# Autodesk Inventor assembly: Touch Segment
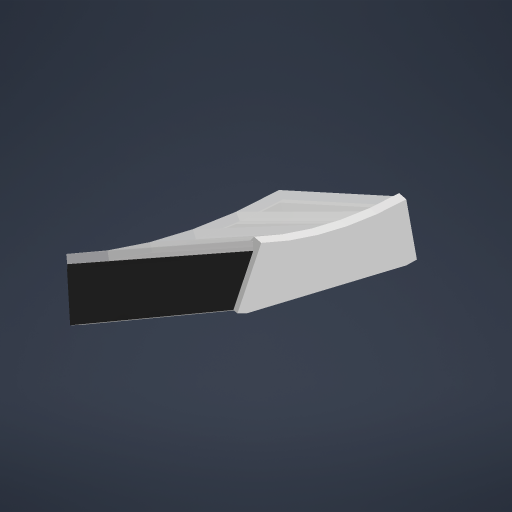
[picture p0: Inventor's stored thumbnail of the model, 512x512]
Saved by Autodesk Inventor 2023 (Build 270158000, 158)
## iProperties
Created: 2022-06-12
Part Number: Touch Segment
Document SubType Name: Assembly
Designer: FizzyApple12
Author: FizzyApple12
## Documents named in this file (4)
- C:\Users\FizzyApple12\Desktop\Wacca Controller\Touch Segment\Touch Segment.iam
- C:\Users\FizzyApple12\Desktop\Wacca Controller\Touch Segment\Touch Fifth.ipt
- C:\Users\FizzyApple12\Desktop\Wacca Controller\Touch Segment\Touch Casing.ipt
- C:\Users\FizzyApple12\Desktop\Wacca Controller\Touch Segment\Touch Segment Cover.ipt
## Components (7 placed, 3 different names)
1. Touch Fifth:1 — Mate:1, Mate:5, Flush:6, Mate:19, Mate:22, Mate:25, Mate:26, Flush:7, Flush:14
2. Touch Fifth:2 — Mate:1, Mate:2, Mate:5, Mate:6, Flush:5, Mate:16, Mate:18, Mate:20, Mate:21, Flush:13
3. Touch Fifth:3 — Mate:2, Mate:3, Mate:6, Mate:7, Mate:8, Flush:1, Flush:2, Mate:13, Mate:15, Mate:17, Flush:12
4. Touch Fifth:4 — Mate:3, Mate:4, Mate:7, Flush:3, Mate:9, Mate:11, Mate:12, Mate:14, Flush:11
5. Touch Fifth:5 — Mate:4, Mate:8, Flush:4, Mate:10, Mate:23, Mate:24, Flush:10
6. Touch Casing:1 — Flush:1, Flush:2, Flush:3, Flush:4, Flush:5, Flush:6, Mate:9, Mate:10, Mate:11, Mate:12, Mate:13, Mate:14, Mate:15, Mate:16, Mate:17, Mate:18, Mate:19, Mate:20, Mate:21, Mate:22, Mate:23, Mate:24, Mate:25, Mate:26, Flush:7, Flush:8, Flush:9
7. Touch Segment Cover:1 — Flush:8, Flush:9, Flush:10, Flush:11, Flush:12, Flush:13, Flush:14
## Relationships (40: Mate 26, Flush 14)
- Mate:1: Touch Fifth:1 ↔ Touch Fifth:2
- Mate:2: Touch Fifth:2 ↔ Touch Fifth:3
- Mate:3: Touch Fifth:3 ↔ Touch Fifth:4
- Mate:4: Touch Fifth:4 ↔ Touch Fifth:5
- Mate:5: Touch Fifth:1 ↔ Touch Fifth:2
- Mate:6: Touch Fifth:2 ↔ Touch Fifth:3
- Mate:7: Touch Fifth:3 ↔ Touch Fifth:4
- Mate:8: Touch Fifth:3 ↔ Touch Fifth:5
- Flush:1: Touch Fifth:3 ↔ Touch Casing:1
- Flush:2: Touch Fifth:3 ↔ Touch Casing:1
- Flush:3: Touch Fifth:4 ↔ Touch Casing:1
- Flush:4: Touch Fifth:5 ↔ Touch Casing:1
- Flush:5: Touch Fifth:2 ↔ Touch Casing:1
- Flush:6: Touch Fifth:1 ↔ Touch Casing:1
- Mate:9: Touch Fifth:4 ↔ Touch Casing:1
- Mate:10: Touch Fifth:5 ↔ Touch Casing:1
- Mate:11: Touch Fifth:4 ↔ Touch Casing:1
- Mate:12: Touch Fifth:4 ↔ Touch Casing:1
- Mate:13: Touch Fifth:3 ↔ Touch Casing:1
- Mate:14: Touch Fifth:4 ↔ Touch Casing:1
- Mate:15: Touch Fifth:3 ↔ Touch Casing:1
- Mate:16: Touch Fifth:2 ↔ Touch Casing:1
- Mate:17: Touch Fifth:3 ↔ Touch Casing:1
- Mate:18: Touch Fifth:2 ↔ Touch Casing:1
- Mate:19: Touch Fifth:1 ↔ Touch Casing:1
- Mate:20: Touch Fifth:2 ↔ Touch Casing:1
- Mate:21: Touch Fifth:2 ↔ Touch Casing:1
- Mate:22: Touch Fifth:1 ↔ Touch Casing:1
- Mate:23: Touch Fifth:5 ↔ Touch Casing:1
- Mate:24: Touch Fifth:5 ↔ Touch Casing:1
- Mate:25: Touch Fifth:1 ↔ Touch Casing:1
- Mate:26: Touch Fifth:1 ↔ Touch Casing:1
- Flush:7: Touch Fifth:1 ↔ Touch Casing:1
- Flush:8: Touch Casing:1 ↔ Touch Segment Cover:1
- Flush:9: Touch Casing:1 ↔ Touch Segment Cover:1
- Flush:10: Touch Fifth:5 ↔ Touch Segment Cover:1
- Flush:11: Touch Fifth:4 ↔ Touch Segment Cover:1
- Flush:12: Touch Fifth:3 ↔ Touch Segment Cover:1
- Flush:13: Touch Fifth:2 ↔ Touch Segment Cover:1
- Flush:14: Touch Fifth:1 ↔ Touch Segment Cover:1
